# Autodesk Inventor assembly: Редуктор в сборе
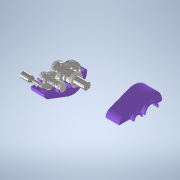
[picture p0: Inventor's stored thumbnail of the model, 180x180]
Saved by Autodesk Inventor 2021 (Build 250183000, 183)
## iProperties
Created: 2023-03-03
Part Number: Редуктор в сборе
Document SubType Name: Assembly
Designer: gdevc
Mass: 9249.32 g
Surface Area: 2771.27 cm^2
Volume: 1186.1 cm^3
Density: 7.79807 g/cm^3
Author: gdevc
## Documents named in this file (16)
- C:\Users\gdevc\OneDrive\Рабочий стол\Курсач\Новая папка\Редуктор в сборе.iam
- C:\Users\gdevc\OneDrive\Рабочий стол\Курсач\Новая папка\Вал_промежуточный.ipt
- C:\Users\gdevc\OneDrive\Рабочий стол\Курсач\Новая папка\Редуктор в сборе\Мастер проектирования\Цилиндрическое зубчатое зацепление1.iam
- C:\Users\gdevc\OneDrive\Рабочий стол\Курсач\Новая папка\Колесо быстроходное.ipt
- C:\Users\gdevc\OneDrive\Рабочий стол\Курсач\Новая папка\Редуктор в сборе\Мастер проектирования\Цилиндрическое зубчатое зацепление2.iam
- C:\Users\gdevc\OneDrive\Рабочий стол\Курсач\Новая папка\Вал_тихоходный.ipt
- C:\Users\gdevc\OneDrive\Рабочий стол\Курсач\Новая папка\Редуктор в сборе\Мастер проектирования\Цилиндрическое зубчатое зацепление3.iam
- C:\Users\gdevc\OneDrive\Рабочий стол\Курсач\Новая папка\Валл быстроходный.ipt
- C:\Users\gdevc\OneDrive\Рабочий стол\Курсач\Новая папка\Редуктор в сборе\Мастер проектирования\Цилиндрическое зубчатое зацепление4.iam
- C:\Users\gdevc\OneDrive\Документы\Inventor\Content Center Files\R2021\GOST 8338-75\Подшипник 205 ГОСТ 8338-75.ipt
- C:\Users\gdevc\OneDrive\Документы\Inventor\Content Center Files\R2021\GOST 8338-75\Подшипник 210 ГОСТ 8338-75.ipt
- C:\Users\gdevc\OneDrive\Документы\Inventor\Content Center Files\R2021\GOST 8752-79(2)\Манжет 2-50x65x8 ГОСТ 8752-79.ipt
- C:\Users\gdevc\OneDrive\Рабочий стол\Курсач\Новая папка\Корпус_v.0.1.iam
- C:\Users\gdevc\OneDrive\Рабочий стол\Курсач\Новая папка\Крышка тих_выход.ipt
- C:\Users\gdevc\OneDrive\Рабочий стол\Курсач\Новая папка\Крышка, тихая.ipt
- C:\Users\gdevc\OneDrive\Рабочий стол\Курсач\Новая папка\Крышка_пром.ipt
## Components (18 placed, 12 different names)
1. Вал_промежуточный:1 — Совмещение:2, Совмещение:4, Совмещение:5, Совмещение:6, Угол:1, Совмещение:9, Заподлицо:2, Совмещение:14, Совмещение:15, Совмещение:16, Совмещение:17, Симметрия:1, Совмещение:25, Совмещение:27
2. Цилиндрическое зубчатое зацепление:1 [sub-assembly]
3. Колесо быстроходное:1 — Совмещение:4, Совмещение:5, Заподлицо:1
4. Цилиндрическое зубчатое зацепление:2 [sub-assembly]
5. Вал_тихоходный:1 — Совмещение:7, Совмещение:8, Совмещение:9, Заподлицо:2, Совмещение:10, Совмещение:11, Совмещение:12, Совмещение:13, Совмещение:18, Совмещение:19, Совмещение:21, Совмещение:23
6. Цилиндрическое зубчатое зацепление:3 [sub-assembly]
7. Валл быстроходный:1 — Совмещение:1, Совмещение:2, Совмещение:6, Заподлицо:1, Угол:1, Совмещение:7, Совмещение:8
8. Цилиндрическое зубчатое зацепление:4 [sub-assembly]
9. Подшипник ГОСТ 8338-75 205:1 — Совмещение:14, Совмещение:15, Симметрия:1, Совмещение:26
10. Подшипник ГОСТ 8338-75 205:2 — Совмещение:16, Совмещение:17, Совмещение:20, Совмещение:28
11. Подшипник ГОСТ 8338-75 210:1 — Совмещение:10, Совмещение:11
12. Подшипник ГОСТ 8338-75 210:2 — Совмещение:12, Совмещение:13
13. Манжет 2 ГОСТ 8752-79 50 x 65 x 8:1 — Совмещение:18
14. Корпус_v.0.1:1 [sub-assembly] — Угол:2, Совмещение:19, Совмещение:20, Совмещение:22, Совмещение:24
15. Крышка тих_выход:1 — Совмещение:21, Совмещение:22
16. Крышка, тихая:1 — Совмещение:23, Совмещение:24
17. Крышка_пром:1 — Совмещение:25, Совмещение:26
18. Крышка_пром:2 — Совмещение:27, Совмещение:28
## Relationships (32: Mate 27, Flush 2, Angle 2, Symmetry 1)
- Совмещение:1 [Mate]: Валл быстроходный:1
- Совмещение:2 [Mate] (63 mm): Вал_промежуточный:1 ↔ Валл быстроходный:1
- Совмещение:4 [Mate]: Вал_промежуточный:1 ↔ Колесо быстроходное:1
- Совмещение:5 [Mate]: Вал_промежуточный:1 ↔ Колесо быстроходное:1
- Совмещение:6 [Mate]: Вал_промежуточный:1 ↔ Валл быстроходный:1
- Заподлицо:1 [Flush] (1 mm): Колесо быстроходное:1 ↔ Валл быстроходный:1
- Угол:1 [Angle] (90 deg): Вал_промежуточный:1 ↔ Валл быстроходный:1
- Совмещение:7 [Mate]: Вал_тихоходный:1 ↔ Валл быстроходный:1
- Совмещение:8 [Mate]: Вал_тихоходный:1 ↔ Валл быстроходный:1
- Совмещение:9 [Mate] (-100 mm): Вал_промежуточный:1 ↔ Вал_тихоходный:1
- Заподлицо:2 [Flush] (1.5 mm): Вал_промежуточный:1 ↔ Вал_тихоходный:1
- Совмещение:10 [Mate]: Вал_тихоходный:1 ↔ Подшипник ГОСТ 8338-75 210:1
- Совмещение:11 [Mate]: Вал_тихоходный:1 ↔ Подшипник ГОСТ 8338-75 210:1
- Совмещение:12 [Mate]: Вал_тихоходный:1 ↔ Подшипник ГОСТ 8338-75 210:2
- Совмещение:13 [Mate]: Вал_тихоходный:1 ↔ Подшипник ГОСТ 8338-75 210:2
- Совмещение:14 [Mate]: Вал_промежуточный:1 ↔ Подшипник ГОСТ 8338-75 205:1
- Совмещение:15 [Mate]: Вал_промежуточный:1 ↔ Подшипник ГОСТ 8338-75 205:1
- Совмещение:16 [Mate]: Вал_промежуточный:1 ↔ Подшипник ГОСТ 8338-75 205:2
- Совмещение:17 [Mate]: Вал_промежуточный:1 ↔ Подшипник ГОСТ 8338-75 205:2
- Совмещение:18 [Mate]: Вал_тихоходный:1 ↔ Манжет 2 ГОСТ 8752-79 50 x 65 x 8:1
- Симметрия:1 [Symmetry]: Вал_промежуточный:1 ↔ Подшипник ГОСТ 8338-75 205:1
- Угол:2 [Angle] (90 deg): Корпус_v.0.1:1
- Совмещение:19 [Mate]: Вал_тихоходный:1 ↔ Корпус_v.0.1:1
- Совмещение:20 [Mate]: Подшипник ГОСТ 8338-75 205:2 ↔ Корпус_v.0.1:1
- Совмещение:21 [Mate]: Вал_тихоходный:1 ↔ Крышка тих_выход:1
- Совмещение:22 [Mate]: Корпус_v.0.1:1 ↔ Крышка тих_выход:1
- Совмещение:23 [Mate]: Вал_тихоходный:1 ↔ Крышка, тихая:1
- Совмещение:24 [Mate]: Корпус_v.0.1:1 ↔ Крышка, тихая:1
- Совмещение:25 [Mate]: Вал_промежуточный:1 ↔ Крышка_пром:1
- Совмещение:26 [Mate]: Подшипник ГОСТ 8338-75 205:1 ↔ Крышка_пром:1
- Совмещение:27 [Mate]: Вал_промежуточный:1 ↔ Крышка_пром:2
- Совмещение:28 [Mate]: Подшипник ГОСТ 8338-75 205:2 ↔ Крышка_пром:2
